# Autodesk Inventor assembly: ArmAssembly
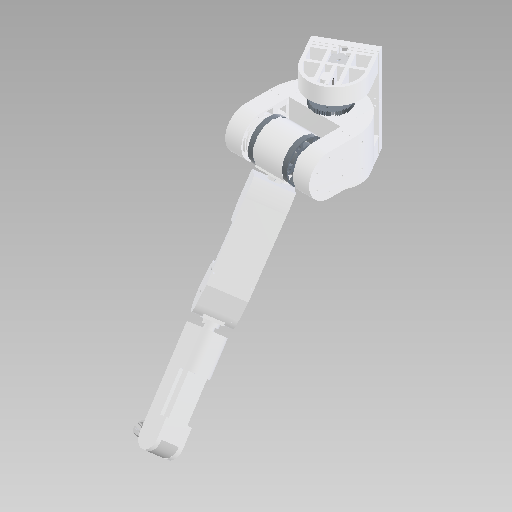
[picture p0: Inventor's stored thumbnail of the model, 512x512]
Saved by Autodesk Inventor 2017 (Build 210142000, 142)
## iProperties
Created: 2017-05-10
Part Number: ArmAssembly
Document SubType Name: Assembly
Designer: zallen
Author: zallen
## Documents named in this file (13)
- C:\Users\zallen\Documents\GitHub\cr-laundry-robot\src\Body\Arm Assembly\ArmAssembly.iam
- C:\Users\zallen\Documents\GitHub\cr-laundry-robot\src\Body\Arm Assembly\Part3.ipt
- C:\Users\zallen\Documents\GitHub\cr-laundry-robot\src\Body\Arm Assembly\Part4.ipt
- C:\Users\zallen\Documents\GitHub\cr-laundry-robot\src\Body\Arm Assembly\Part5.ipt
- C:\Users\zallen\Documents\GitHub\cr-laundry-robot\src\Body\Arm Assembly\Part6.ipt
- C:\Users\zallen\Documents\GitHub\cr-laundry-robot\src\Body\Arm Assembly\Part7.ipt
- C:\Users\zallen\Documents\GitHub\cr-laundry-robot\src\Body\Arm Assembly\Part8.ipt
- C:\Users\zallen\Documents\GitHub\cr-laundry-robot\lib\Stepper Motor\Двигатель.ipt
- C:\Users\zallen\Documents\GitHub\cr-laundry-robot\src\Body\Arm Assembly\ArmAssembly\Design Accelerator\Spur Gears2.iam
- C:\Users\zallen\Documents\GitHub\cr-laundry-robot\src\Body\Arm Assembly\Part10.ipt
- C:\Users\zallen\Documents\GitHub\cr-laundry-robot\src\Body\Arm Assembly\Part11.ipt
- C:\Users\zallen\Documents\GitHub\cr-laundry-robot\src\Body\Arm Assembly\Part12.ipt
- C:\Users\zallen\Documents\GitHub\cr-laundry-robot\src\Body\Arm Assembly\Shoulder Joint Assembly\Shoulder Joint Assembly.iam
## Components (15 placed, 12 different names)
1. Part3:1 — Mate:39, Rotational:16, Mate:41, Mate:42, Mate:43, Mate:47, Mate:51, Mate:52, Mate:55, Mate:56, Mate:57, Mate:58, Mate:59, Mate:60, Mate:61, Mate:62, Mate:66, Mate:70
2. Part4:1 — Mate:39, Mate:40, Rotational:15, Rotational:16
3. Part5:1 — Mate:8, Rotational:8, Mate:40, Rotational:15
4. Part6:1 — Mate:8, Mate:9, Rotational:8, Rotational:9
5. Part7:1 — Mate:9, Rotational:9, Mate:10, Rotational:10, Mate:11, Rotational:11
6. Part8:1 — Mate:10, Rotational:10
7. Part8:2 — Mate:11, Rotational:11
8. Двигатель:2 — Mate:63, Mate:64
9. Двигатель:4 — Mate:41, Mate:42, Mate:43, Mate:46
10. Spur Gears:1 [sub-assembly] — Mate:46, Mate:47
11. Part10:1 — Mate:51, Mate:54
12. Part11:1 — Mate:52, Mate:54, Mate:55, Mate:56
13. Part11:2 — Mate:57, Mate:58, Mate:59
14. Part12:1 — Mate:60, Mate:61, Mate:62
15. Shoulder Joint Assembly:1 [sub-assembly] — Mate:63, Mate:64, Mate:66, Mate:67, Mate:68, Mate:69, Mate:70
## Relationships (35: Mate 29, RevoluteJoint 6)
- Mate:8: Part5:1 ↔ Part6:1
- Mate:9: Part6:1 ↔ Part7:1
- Rotational:8 [RevoluteJoint]: Part5:1 ↔ Part6:1
- Rotational:9 [RevoluteJoint]: Part6:1 ↔ Part7:1
- Mate:10: Part7:1 ↔ Part8:1
- Rotational:10 [RevoluteJoint]: Part7:1 ↔ Part8:1
- Mate:11: Part7:1 ↔ Part8:2
- Rotational:11 [RevoluteJoint]: Part7:1 ↔ Part8:2
- Mate:39: Part3:1 ↔ Part4:1
- Mate:40: Part4:1 ↔ Part5:1
- Rotational:15 [RevoluteJoint]: Part4:1 ↔ Part5:1
- Rotational:16 [RevoluteJoint]: Part3:1 ↔ Part4:1
- Mate:41: Part3:1 ↔ Двигатель:4
- Mate:42: Part3:1 ↔ Двигатель:4
- Mate:43: Part3:1 ↔ Двигатель:4
- Mate:46: Двигатель:4 ↔ Spur Gears:1
- Mate:47: Part3:1 ↔ Spur Gears:1
- Mate:51: Part3:1 ↔ Part10:1
- Mate:52: Part3:1 ↔ Part11:1
- Mate:54: Part10:1 ↔ Part11:1
- Mate:55: Part3:1 ↔ Part11:1
- Mate:56: Part3:1 ↔ Part11:1
- Mate:57: Part3:1 ↔ Part11:2
- Mate:58: Part3:1 ↔ Part11:2
- Mate:59: Part3:1 ↔ Part11:2
- Mate:60: Part3:1 ↔ Part12:1
- Mate:61: Part3:1 ↔ Part12:1
- Mate:62: Part3:1 ↔ Part12:1
- Mate:63: Двигатель:2 ↔ Shoulder Joint Assembly:1
- Mate:64: Двигатель:2 ↔ Shoulder Joint Assembly:1
- Mate:66: Part3:1 ↔ Shoulder Joint Assembly:1
- Mate:67: Shoulder Joint Assembly:1
- Mate:68: Shoulder Joint Assembly:1
- Mate:69: Shoulder Joint Assembly:1
- Mate:70: Part3:1 ↔ Shoulder Joint Assembly:1
